# Autodesk Inventor assembly: EngineAssemblyNEW
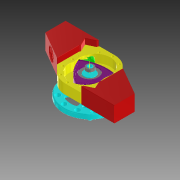
[picture p0: Inventor's stored thumbnail of the model, 180x180]
Saved by Autodesk Inventor 2020 (Build 240168000, 168)
## iProperties
Created: 2021-02-15
Part Number: EngineAssemblyNEW
Document SubType Name: Assembly
Designer: DDeGo
Author: DDeGo
## Documents named in this file (15)
- C:\Users\DDeGo\Documents\Drew\Projects\AirWankelEngine\cad\Wankel V1\EngineAssembly.iam
- C:\Users\DDeGo\Documents\Drew\Projects\AirWankelEngine\cad\Wankel V1\housing.ipt
- C:\Users\DDeGo\Documents\Drew\Projects\AirWankelEngine\cad\Wankel V1\housingValve.ipt
- C:\Users\DDeGo\Documents\Drew\Projects\AirWankelEngine\cad\Wankel V1\ValveFlapper.ipt
- C:\Users\DDeGo\Documents\Drew\Projects\AirWankelEngine\cad\Wankel V1\housingPlate.ipt
- C:\Users\DDeGo\Documents\Drew\Projects\AirWankelEngine\cad\Wankel V1\piston.ipt
- C:\Users\DDeGo\Documents\Drew\Projects\AirWankelEngine\cad\hardware\6701 bearing.ipt
- C:\Users\DDeGo\Documents\Drew\Projects\AirWankelEngine\cad\hardware\MR85 bearing.ipt
- C:\Users\DDeGo\Documents\Drew\Projects\AirWankelEngine\cad\Wankel V1\camshaft.ipt
- C:\Users\DDeGo\Documents\Drew\Projects\AirWankelEngine\cad\Wankel V1\CamPlate.ipt
- C:\Users\DDeGo\Documents\Drew\Projects\AirWankelEngine\cad\Wankel V1\Flywheel.ipt
- C:\Users\DDeGo\Documents\Drew\Projects\AirWankelEngine\cad\hardware\oring_4x8.ipt
- C:\Users\DDeGo\Documents\Drew\Projects\AirWankelEngine\cad\hardware\6mm bb.ipt
- C:\Users\DDeGo\Documents\Drew\Projects\AirWankelEngine\cad\Wankel V1\proto_clamp.ipt
- C:\Users\DDeGo\Documents\Drew\Projects\AirWankelEngine\cad\hardware\ApexSeal_oring_2mm.ipt
## Components (23 placed, 14 different names)
1. housing:1 — Mate:1, Mate:2, Mate:3, Mate:4, Mate:5, Mate:6, Mate:7, Mate:8, Mate:9, Mate:10, Mate:14, Mate:15, Mate:16, Mate:17, Mate:29, Mate:32, Mate:44
2. housingValve:1 — Mate:1, Mate:5, Mate:6, Mate:35, Mate:36, Flush:2, Mate:38, Mate:39
3. ValveFlapper:1 — Mate:7, Mate:8, Flush:1
4. housingValve:2 — Mate:2, Mate:3, Mate:4, Mate:30, Mate:31, Mate:33, Mate:40
5. housingPlate:1 — Mate:9, Mate:10, Mate:22, Mate:44
6. piston:1 — Mate:12, Mate:13, Mate:14, Rotation:1, Flush:5, Mate:41, Mate:42, Mate:43
7. 6701 bearing:1 — Mate:12, Mate:13, Mate:18
8. MR85 bearing:1 — Mate:15, Mate:16, Mate:19
9. camshaft:1 — Mate:17, Mate:18, Mate:19, Mate:21, Mate:23, Mate:26, Mate:28, Rotation:1
10. MR85 bearing:2 — Mate:21, Mate:22
11. CamPlate:1 — Mate:23, Mate:24, Mate:25, Mate:26, Mate:27, Mate:28
12. Flywheel:1 — Mate:24, Mate:25, Mate:27
13. ValveFlapper:2 — Mate:29, Flush:1
14. oring_4x8:1 — Mate:30, Mate:31, Mate:34
15. oring_4x8:2 — Mate:36, Flush:2
16. oring_4x8:3 — Mate:35, Mate:37, Mate:38
17. oring_4x8:4 — Mate:32, Mate:33
18. 6mm bb:1 — Mate:34
19. 6mm bb:2 — Mate:37
20. proto_clamp:1 — Mate:39, Mate:40
21. ApexSeal_oring_2mm:1 — Flush:3, Flush:4, Flush:5, Mate:41
22. ApexSeal_oring_2mm:2 — Flush:3, Mate:42
23. ApexSeal_oring_2mm:3 — Flush:4, Mate:43
## Relationships (48: Mate 42, Flush 5, RelateRotation 1)
- Mate:1: housing:1 ↔ housingValve:1
- Mate:2: housing:1 ↔ housingValve:2
- Mate:3: housing:1 ↔ housingValve:2
- Mate:4: housing:1 ↔ housingValve:2
- Mate:5: housing:1 ↔ housingValve:1
- Mate:6: housing:1 ↔ housingValve:1
- Mate:7: housing:1 ↔ ValveFlapper:1
- Mate:8 (0.2 mm): housing:1 ↔ ValveFlapper:1
- Mate:9: housing:1 ↔ housingPlate:1
- Mate:10: housing:1 ↔ housingPlate:1
- Mate:12: piston:1 ↔ 6701 bearing:1
- Mate:13: piston:1 ↔ 6701 bearing:1
- Mate:14 (0.2 mm): housing:1 ↔ piston:1
- Mate:15: housing:1 ↔ MR85 bearing:1
- Mate:16: housing:1 ↔ MR85 bearing:1
- Mate:17: housing:1 ↔ camshaft:1
- Mate:18: 6701 bearing:1 ↔ camshaft:1
- Mate:19: MR85 bearing:1 ↔ camshaft:1
- Mate:21: camshaft:1 ↔ MR85 bearing:2
- Mate:22: housingPlate:1 ↔ MR85 bearing:2
- Mate:23: camshaft:1 ↔ CamPlate:1
- Mate:24: CamPlate:1 ↔ Flywheel:1
- Mate:25: CamPlate:1 ↔ Flywheel:1
- Mate:26: camshaft:1 ↔ CamPlate:1
- Mate:27: CamPlate:1 ↔ Flywheel:1
- Mate:28: camshaft:1 ↔ CamPlate:1
- Rotation:1 [RelateRotation] (3 ul): piston:1 ↔ camshaft:1
- Mate:29: housing:1 ↔ ValveFlapper:2
- Flush:1: ValveFlapper:1 ↔ ValveFlapper:2
- Mate:30: housingValve:2 ↔ oring_4x8:1
- Mate:31: housingValve:2 ↔ oring_4x8:1
- Mate:32: housing:1 ↔ oring_4x8:4
- Mate:33: housingValve:2 ↔ oring_4x8:4
- Mate:34: oring_4x8:1 ↔ 6mm bb:1
- Mate:35: housingValve:1 ↔ oring_4x8:3
- Mate:36: housingValve:1 ↔ oring_4x8:2
- Mate:37: oring_4x8:3 ↔ 6mm bb:2
- Flush:2: housingValve:1 ↔ oring_4x8:2
- Mate:38: housingValve:1 ↔ oring_4x8:3
- Mate:39: housingValve:1 ↔ proto_clamp:1
- Mate:40: housingValve:2 ↔ proto_clamp:1
- Flush:3: ApexSeal_oring_2mm:1 ↔ ApexSeal_oring_2mm:2
- Flush:4: ApexSeal_oring_2mm:1 ↔ ApexSeal_oring_2mm:3
- Flush:5: piston:1 ↔ ApexSeal_oring_2mm:1
- Mate:41: piston:1 ↔ ApexSeal_oring_2mm:1
- Mate:42: piston:1 ↔ ApexSeal_oring_2mm:2
- Mate:43: piston:1 ↔ ApexSeal_oring_2mm:3
- Mate:44: housing:1 ↔ housingPlate:1
